# Autodesk Inventor assembly: StrainWaveGearbox
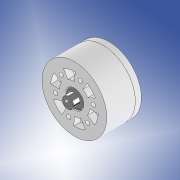
[picture p0: Inventor's stored thumbnail of the model, 180x180]
Saved by Autodesk Inventor 2017 SP1 (Build 210196100, 196)
## iProperties
Created: 2017-07-11
Part Number: StrainWaveGearbox
Document SubType Name: Assembly
Designer: zallen
Author: zallen
## Documents named in this file (12)
- C:\Users\Zach\Documents\GitHub\cr-laundry-robot\lib\Strain Wave Gearbox 12_1\StrainWaveGearbox_12_1.iam
- C:\Users\Zach\Documents\GitHub\cr-laundry-robot\lib\Strain Wave Gearbox 12_1\Flexspline.ipt
- C:\Users\Zach\Documents\GitHub\cr-laundry-robot\lib\Strain Wave Gearbox 12_1\Basespline.ipt
- C:\Users\Zach\Documents\GitHub\cr-laundry-robot\lib\Strain Wave Gearbox 12_1\WaveGenerator.ipt
- C:\Users\Zach\Documents\GitHub\cr-laundry-robot\lib\Strain Wave Gearbox 12_1\FlexsplineCover.ipt
- C:\Users\Zach\Documents\GitHub\cr-laundry-robot\lib\Strain Wave Gearbox 12_1\22x8x8mm Bearing.ipt
- C:\Users\Zach\Documents\GitHub\cr-laundry-robot\lib\Strain Wave Gearbox 12_1\WaveGeneratorRoller.ipt
- C:\Users\Zach\Documents\GitHub\cr-laundry-robot\lib\Strain Wave Gearbox 12_1\WaveGeneratorCover.ipt
- C:\Users\Zach\Documents\GitHub\cr-laundry-robot\lib\ISO 7091 - ST 8 - 100 HV.ipt
- C:\Users\Zach\Documents\GitHub\cr-laundry-robot\lib\CNS 3129 - M 8 x 1.25.ipt
- C:\Users\Zach\Documents\GitHub\cr-laundry-robot\lib\CNS 3932 - M 8 x 1.25 x 40.ipt
- C:\Users\Zach\Documents\GitHub\cr-laundry-robot\lib\13x4x5mm Bearing.ipt
## Components (17 placed, 11 different names)
1. Flexspline:1 — Mate:1, Mate:6, Mate:9, Mate:10, Mate:38
2. Basespline:1 — Mate:1, Flush:2, Mate:2, Mate:3, Mate:4, Rotation:1, Mate:6, Mate:7, Flush:3, Mate:37
3. WaveGenerator:1 — Mate:4, Rotation:1, Mate:17, Mate:20, Mate:21, Mate:22, Mate:33, Rotation:2, Mate:46, Mate:47, Mate:48, Mate:49, Mate:51, Mate:52
4. FlexsplineCover:1 — Mate:9, Mate:10, Mate:11, Mate:37, Mate:38
5. 22x8x8mm Bearing:1 — Mate:7, Flush:3, Mate:34, Mate:35, Mate:40
6. 22x8x8mm Bearing:2 — Mate:11, Mate:28
7. WaveGeneratorRoller:1 — Mate:17, Mate:50
8. WaveGeneratorRoller:2 — Mate:20, Mate:21
9. WaveGeneratorCover:1 — Mate:22, Mate:51, Mate:52
10. ISO 7091 ST 8 - 100 HV:1 — Mate:43, Mate:45
11. CNS 3129 M 8:1 — Mate:28, Mate:36
12. ISO 7091 ST 8 - 100 HV:2 — Mate:33, Mate:41, Mate:42
13. CNS 3932 M 8 x 40:1 — Mate:34, Mate:35, Mate:36, Rotation:2, Mate:39, Mate:42, Mate:43, Mate:44
14. ISO 7091 ST 8 - 100 HV:3 — Mate:44, Mate:45
15. ISO 7091 ST 8 - 100 HV:4 — Mate:39, Mate:40, Mate:41
16. 13x4x5mm Bearing:1 — Mate:46, Mate:47, Mate:50
17. 13x4x5mm Bearing:2 — Mate:48, Mate:49
## Relationships (38: Mate 34, Flush 2, RelateRotation 2)
- Mate:1: Flexspline:1 ↔ Basespline:1
- Flush:2: Basespline:1
- Mate:2: Basespline:1
- Mate:3: Basespline:1
- Mate:4: Basespline:1 ↔ WaveGenerator:1
- Rotation:1 [RelateRotation] (0.0217 ul): Basespline:1 ↔ WaveGenerator:1
- Mate:6: Flexspline:1 ↔ Basespline:1
- Mate:7: Basespline:1 ↔ 22x8x8mm Bearing:1
- Flush:3: Basespline:1 ↔ 22x8x8mm Bearing:1
- Mate:9: Flexspline:1 ↔ FlexsplineCover:1
- Mate:10: Flexspline:1 ↔ FlexsplineCover:1
- Mate:11: FlexsplineCover:1 ↔ 22x8x8mm Bearing:2
- Mate:17: WaveGenerator:1 ↔ WaveGeneratorRoller:1
- Mate:20: WaveGenerator:1 ↔ WaveGeneratorRoller:2
- Mate:21: WaveGenerator:1 ↔ WaveGeneratorRoller:2
- Mate:22: WaveGenerator:1 ↔ WaveGeneratorCover:1
- Mate:28: 22x8x8mm Bearing:2 ↔ CNS 3129 M 8:1
- Mate:33: WaveGenerator:1 ↔ ISO 7091 ST 8 - 100 HV:2
- Mate:34: 22x8x8mm Bearing:1 ↔ CNS 3932 M 8 x 40:1
- Mate:35: 22x8x8mm Bearing:1 ↔ CNS 3932 M 8 x 40:1
- Mate:36: CNS 3129 M 8:1 ↔ CNS 3932 M 8 x 40:1
- Rotation:2 [RelateRotation] (1 ul): WaveGenerator:1 ↔ CNS 3932 M 8 x 40:1
- Mate:37: Basespline:1 ↔ FlexsplineCover:1
- Mate:38: Flexspline:1 ↔ FlexsplineCover:1
- Mate:39: CNS 3932 M 8 x 40:1 ↔ ISO 7091 ST 8 - 100 HV:4
- Mate:40: 22x8x8mm Bearing:1 ↔ ISO 7091 ST 8 - 100 HV:4
- Mate:41: ISO 7091 ST 8 - 100 HV:2 ↔ ISO 7091 ST 8 - 100 HV:4
- Mate:42: ISO 7091 ST 8 - 100 HV:2 ↔ CNS 3932 M 8 x 40:1
- Mate:43: ISO 7091 ST 8 - 100 HV:1 ↔ CNS 3932 M 8 x 40:1
- Mate:44: CNS 3932 M 8 x 40:1 ↔ ISO 7091 ST 8 - 100 HV:3
- Mate:45: ISO 7091 ST 8 - 100 HV:1 ↔ ISO 7091 ST 8 - 100 HV:3
- Mate:46: WaveGenerator:1 ↔ 13x4x5mm Bearing:1
- Mate:47: WaveGenerator:1 ↔ 13x4x5mm Bearing:1
- Mate:48: WaveGenerator:1 ↔ 13x4x5mm Bearing:2
- Mate:49: WaveGenerator:1 ↔ 13x4x5mm Bearing:2
- Mate:50: WaveGeneratorRoller:1 ↔ 13x4x5mm Bearing:1
- Mate:51: WaveGenerator:1 ↔ WaveGeneratorCover:1
- Mate:52: WaveGenerator:1 ↔ WaveGeneratorCover:1
